# Autodesk Inventor assembly: SideUndamaged
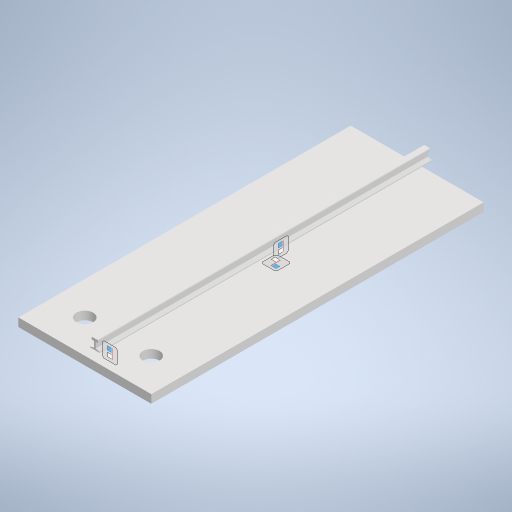
[picture p0: Inventor's stored thumbnail of the model, 512x512]
Saved by Autodesk Inventor 2023 (Build 270158030, 158C)
## iProperties
Created: 2023-02-14
Part Number: SideUndamaged
Document SubType Name: Assembly
Designer: jeremyy
Author: jeremyy
## Documents named in this file (3)
- \\andrew.ad.cmu.edu\users\users1\jeremyy\Documents\Inventor\CMU Bridge\New folder\Figs\SideDamaged.iam
- \\andrew.ad.cmu.edu\users\users1\jeremyy\Documents\Inventor\CMU Bridge\New folder\Figs\Plate2inxShort.ipt
- \\andrew.ad.cmu.edu\users\users1\jeremyy\Documents\Inventor\CMU Bridge\New folder\Figs\RailShort.ipt
## Components (2 placed, 2 different names)
1. Plate2inxShort:1 — Mate:1, Flush:1, Flush:2
2. RailShort:1 — Mate:1, Flush:1, Flush:2
## Relationships (3: Flush 2, Mate 1)
- Mate:1: Plate2inxShort:1 ↔ RailShort:1
- Flush:1 (3.81 mm): Plate2inxShort:1 ↔ RailShort:1
- Flush:2 (23.5458 mm): Plate2inxShort:1 ↔ RailShort:1
